# Autodesk Inventor assembly: Third Extension of Base
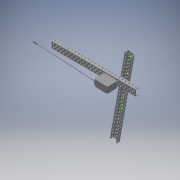
[picture p0: Inventor's stored thumbnail of the model, 180x180]
Saved by Autodesk Inventor 2018 (Build 220112000, 112)
## iProperties
Created: 2017-06-28
Part Number: Third Extension of Base
Document SubType Name: Assembly
Designer: James
Author: James
## Documents named in this file (3)
- C:\Users\James\Desktop\EE REU\Hardware\Vex Arm\Third Extension of Base.iam
- C:\Users\James\Desktop\EE REU\Hardware\Vex Arm\Vex Parts\C_Channel.ipt
- C:\Users\James\Desktop\EE REU\Hardware\Vex Arm\Vex Parts\393motor.ipt
## Components (3 placed, 2 different names)
1. C_Channel:1 — Insert:1
2. C_Channel:2 — Insert:2
3. 393motor:1 — Insert:1, Insert:2
## Relationships (2: Insert 2)
- Insert:1: C_Channel:1 ↔ 393motor:1
- Insert:2 (50 mm): C_Channel:2 ↔ 393motor:1
